# Autodesk Inventor assembly: gate_and
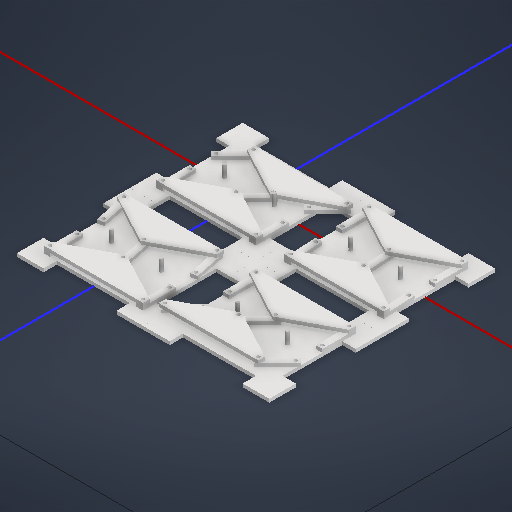
[picture p0: Inventor's stored thumbnail of the model, 512x512]
Saved by Autodesk Inventor 2025.4 (Build 294407000, 407)
## iProperties
Created: 2026-09-12
Part Number: gate_and
Document SubType Name: Assembly
Designer: User
Author: User
## Documents named in this file (2)
- G:\projects\secondary\computer_mechanical\gates\gate_and.iam
- G:\projects\secondary\computer_mechanical\gates\lock\lock.iam
## Components (4 placed, 1 different names)
1. lock:1 [sub-assembly] — Flush:1, Flush:4, Mate:1, Mate:3, Flush:6
2. lock:2 [sub-assembly] — Flush:2, Flush:5, Mate:2
3. lock:3 [sub-assembly] — Flush:1, Flush:2, Flush:3, Flush:4, Mate:1, Flush:5, Mate:2
4. lock:4 [sub-assembly] — Flush:3, Mate:3, Flush:6
## Relationships (9: Flush 6, Mate 3)
- Flush:1: lock:1 ↔ lock:3
- Flush:2: lock:2 ↔ lock:3
- Flush:3: lock:3 ↔ lock:4
- Flush:4: lock:1 ↔ lock:3
- Mate:1: lock:1 ↔ lock:3
- Flush:5: lock:2 ↔ lock:3
- Mate:2: lock:2 ↔ lock:3
- Mate:3: lock:1 ↔ lock:4
- Flush:6: lock:1 ↔ lock:4
